# Autodesk Inventor assembly: FrontCover
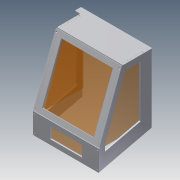
[picture p0: Inventor's stored thumbnail of the model, 180x180]
Saved by Autodesk Inventor 2014 (Build 180170000, 170)
## iProperties
Created: 2014-08-11
Part Number: FrontCover
Document SubType Name: Assembly
Designer: Peele
Author: Peele
## Documents named in this file (9)
- E:\Copy\DLP\DMP-SL-v2\SubAssem\FrontCover.iam
- E:\Copy\DLP\DMP-SL-v2\CustomParts\TopSidePanel.ipt
- E:\Copy\DLP\DMP-SL-v2\CustomParts\TopTopPanel.ipt
- E:\Copy\DLP\DMP-SL-v2\CustomParts\TopFrontPanel.ipt
- E:\Copy\DLP\DMP-SL-v2\CustomParts\TopDiagonalPanel.ipt
- E:\Copy\DLP\DMP-SL-v2\CustomParts\AcrylicDiagonal.ipt
- E:\Copy\DLP\DMP-SL-v2\CustomParts\AcrylicSide.ipt
- E:\Copy\DLP\DMP-SL-v2\CustomParts\AcrylicLogo.ipt
- E:\Copy\DLP\DMP-SL-v2\CustomParts\TopSidePanel-Left.ipt
## Components (9 placed, 8 different names)
1. TopSidePanel:2 — Mate:1, Mate:2, Mate:3, Mate:4, Mate:5, Mate:6, Mate:10, Mate:15, Mate:20, Mate:21
2. TopTopPanel:1 — Mate:4, Mate:5, Mate:6, Mate:19
3. TopFrontPanel:1 — Mate:1, Mate:2, Mate:3, Mate:16, Mate:17, Mate:18
4. TopDiagonalPanel:1 — Mate:10, Mate:13, Mate:20, Mate:21
5. AcrylicDiagonal:1 — Mate:13
6. AcrylicSide:2 — Mate:15
7. AcrylicLogo:1 — Mate:16
8. TopSidePanel-Left:1 — Mate:17, Mate:18, Mate:19, Mate:22
9. AcrylicSide:3 — Mate:22
## Relationships (16: Mate 16)
- Mate:1: TopSidePanel:2 ↔ TopFrontPanel:1
- Mate:2: TopSidePanel:2 ↔ TopFrontPanel:1
- Mate:3: TopSidePanel:2 ↔ TopFrontPanel:1
- Mate:4: TopSidePanel:2 ↔ TopTopPanel:1
- Mate:5: TopSidePanel:2 ↔ TopTopPanel:1
- Mate:6: TopSidePanel:2 ↔ TopTopPanel:1
- Mate:10: TopSidePanel:2 ↔ TopDiagonalPanel:1
- Mate:13: TopDiagonalPanel:1 ↔ AcrylicDiagonal:1
- Mate:15: TopSidePanel:2 ↔ AcrylicSide:2
- Mate:16: TopFrontPanel:1 ↔ AcrylicLogo:1
- Mate:17: TopFrontPanel:1 ↔ TopSidePanel-Left:1
- Mate:18: TopFrontPanel:1 ↔ TopSidePanel-Left:1
- Mate:19: TopTopPanel:1 ↔ TopSidePanel-Left:1
- Mate:20: TopSidePanel:2 ↔ TopDiagonalPanel:1
- Mate:21: TopSidePanel:2 ↔ TopDiagonalPanel:1
- Mate:22: TopSidePanel-Left:1 ↔ AcrylicSide:3
